# Autodesk Inventor assembly: ExtruderSatoerMirrored
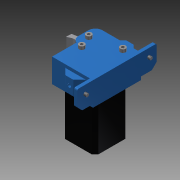
[picture p0: Inventor's stored thumbnail of the model, 180x180]
Saved by Autodesk Inventor 2015 SP1 (Build 190203100, 203)
## iProperties
Created: 2015-05-03
Part Number: ExtruderSatoerMirrored
Document SubType Name: Assembly
Designer: Jack
Author: Jack
## Documents named in this file (13)
- C:\Users\Jack\ownCloud\Projects\CrossBot\InventorModel\Extruder\ExtruderSatoer\ExtruderSatoerLeft\ExtruderSatoerLeft.iam
- C:\Users\Jack\ownCloud\Projects\CrossBot\InventorModel\Extruder\ExtruderSatoer\ExtruderSatoerLeft\ExtruderSatoerBodyLeft.ipt
- C:\Users\Jack\ownCloud\Projects\CrossBot\InventorModel\Extruder\ExtruderSatoer\ExtruderSatoerLeft\ExtruderSatoerMotorMountLeft.ipt
- C:\Users\Jack\ownCloud\Projects\CrossBot\InventorModel\Hardware\Bolts\SHCS\SHCS4\SHCS4x30.ipt
- C:\Users\Jack\ownCloud\Projects\CrossBot\InventorModel\Extruder\ExtruderSatoer\ExtruderSatoerLeft\ExtruderSatoerBearingArmLeft.ipt
- C:\Users\Jack\ownCloud\Projects\CrossBot\InventorModel\Extruder\ExtruderSatoer\ExtruderSatoerLeft\ExtruderSatoerCamLeft.ipt
- C:\Users\Jack\ownCloud\Projects\CrossBot\InventorModel\Extruder\ExtruderSatoer\ExtruderSatoerLeft\ExtruderSatoerCamArmLeft.ipt
- C:\Users\Jack\ownCloud\Projects\CrossBot\InventorModel\Hardware\Bearing\BearingRadialBall\BearingRadialBall624zz.ipt
- C:\Users\Jack\ownCloud\Projects\CrossBot\InventorModel\Hardware\Bolts\SHCS\SHCS4\SHCS4x12.ipt
- C:\Users\Jack\ownCloud\Projects\CrossBot\InventorModel\Hardware\Nuts\Nut4.ipt
- C:\Users\Jack\ownCloud\Projects\CrossBot\InventorModel\Hardware\BoltWashers\BoltWasher4\BoltWasher4x8.iam
- C:\Users\Jack\ownCloud\Projects\CrossBot\InventorModel\Hardware\Bolts\SHCS\SHCS3\SHCS3x12.ipt
- C:\Users\Jack\ownCloud\Projects\CrossBot\InventorModel\Electronics\Motors\StepperMotorNema17x60mm.ipt
## Components (21 placed, 12 different names)
1. ExtruderSatoerBodyLeft:1 — Mate:3, Mate:2, Mate:1, Mate:8, Mate:6, Mate:7, Mate:5, Mate:9, Mate:4, Mate:13, Mate:16, Mate:15, Mate:25, Mate:22, Mate:24, Mate:23
2. ExtruderSatoerMotorMountLeft:1 — Mate:3, Mate:2, Mate:1, Angle:2, Mate:31, Angle:3, Mate:30, Angle:4, Mate:29, Mate:37, Mate:34, Mate:39, Mate:33, Mate:36, Mate:35, Mate:38, Mate:32, Mate:42, Mate:40
3. SHCS4x30:1 — Mate:8, Mate:6, Mate:14, Mate:28
4. SHCS4x30:2 — Mate:7, Mate:5, Mate:12, Mate:26
5. SHCS4x30:3 — Mate:9, Mate:4, Mate:17, Mate:27
6. ExtruderSatoerBearingArmLeft:1 — Mate:13, Mate:12, Mate:11, Mate:10, Mate:19, Mate:18, Mate:21, Angle:1
7. ExtruderSatoerCamLeft:1 — Mate:17, Mate:16
8. ExtruderSatoerCamArmLeft:1 — Mate:15, Mate:14
9. BearingRadialBall624zz:1 — Mate:11, Mate:10
10. SHCS4x12:1 — Mate:19, Mate:18, Mate:20
11. Nut4:1 — Mate:21, Angle:1, Mate:20
12. BoltWasher4x8:1 [sub-assembly] — Mate:25, Mate:22
13. BoltWasher4x8:2 [sub-assembly] — Mate:24, Mate:23
14. Nut4:2 — Angle:2, Mate:31, Mate:26
15. Nut4:3 — Angle:3, Mate:30, Mate:27
16. Nut4:4 — Angle:4, Mate:29, Mate:28
17. SHCS3x12:1 — Mate:37, Mate:34
18. SHCS3x12:2 — Mate:39, Mate:33
19. SHCS3x12:3 — Mate:36, Mate:35
20. SHCS3x12:4 — Mate:38, Mate:32, Mate:41
21. StepperMotorNema17x60mm:1 — Mate:42, Mate:41, Mate:40
## Relationships (46: Mate 42, Angle 4)
- Mate:3: ExtruderSatoerBodyLeft:1 ↔ ExtruderSatoerMotorMountLeft:1
- Mate:2 (0.25 mm): ExtruderSatoerBodyLeft:1 ↔ ExtruderSatoerMotorMountLeft:1
- Mate:1 (0.25 mm): ExtruderSatoerBodyLeft:1 ↔ ExtruderSatoerMotorMountLeft:1
- Mate:8: ExtruderSatoerBodyLeft:1 ↔ SHCS4x30:1
- Mate:6: ExtruderSatoerBodyLeft:1 ↔ SHCS4x30:1
- Mate:7: ExtruderSatoerBodyLeft:1 ↔ SHCS4x30:2
- Mate:5: ExtruderSatoerBodyLeft:1 ↔ SHCS4x30:2
- Mate:9: ExtruderSatoerBodyLeft:1 ↔ SHCS4x30:3
- Mate:4: ExtruderSatoerBodyLeft:1 ↔ SHCS4x30:3
- Mate:13 (0.15 mm): ExtruderSatoerBodyLeft:1 ↔ ExtruderSatoerBearingArmLeft:1
- Mate:12: SHCS4x30:2 ↔ ExtruderSatoerBearingArmLeft:1
- Mate:17: SHCS4x30:3 ↔ ExtruderSatoerCamLeft:1
- Mate:16 (0.15 mm): ExtruderSatoerBodyLeft:1 ↔ ExtruderSatoerCamLeft:1
- Mate:15 (0.15 mm): ExtruderSatoerBodyLeft:1 ↔ ExtruderSatoerCamArmLeft:1
- Mate:14: SHCS4x30:1 ↔ ExtruderSatoerCamArmLeft:1
- Mate:11: ExtruderSatoerBearingArmLeft:1 ↔ BearingRadialBall624zz:1
- Mate:10: ExtruderSatoerBearingArmLeft:1 ↔ BearingRadialBall624zz:1
- Mate:19: ExtruderSatoerBearingArmLeft:1 ↔ SHCS4x12:1
- Mate:18: ExtruderSatoerBearingArmLeft:1 ↔ SHCS4x12:1
- Mate:21: ExtruderSatoerBearingArmLeft:1 ↔ Nut4:1
- Angle:1 (0 deg): ExtruderSatoerBearingArmLeft:1 ↔ Nut4:1
- Mate:20: SHCS4x12:1 ↔ Nut4:1
- Mate:25: ExtruderSatoerBodyLeft:1 ↔ BoltWasher4x8:1
- Mate:22: ExtruderSatoerBodyLeft:1 ↔ BoltWasher4x8:1
- Mate:24: ExtruderSatoerBodyLeft:1 ↔ BoltWasher4x8:2
- Mate:23: ExtruderSatoerBodyLeft:1 ↔ BoltWasher4x8:2
- Angle:2 (0 deg): ExtruderSatoerMotorMountLeft:1 ↔ Nut4:2
- Mate:31: ExtruderSatoerMotorMountLeft:1 ↔ Nut4:2
- Mate:26: SHCS4x30:2 ↔ Nut4:2
- Angle:3 (0 deg): ExtruderSatoerMotorMountLeft:1 ↔ Nut4:3
- Mate:30: ExtruderSatoerMotorMountLeft:1 ↔ Nut4:3
- Mate:27: SHCS4x30:3 ↔ Nut4:3
- Angle:4 (0 deg): ExtruderSatoerMotorMountLeft:1 ↔ Nut4:4
- Mate:29: ExtruderSatoerMotorMountLeft:1 ↔ Nut4:4
- Mate:28: SHCS4x30:1 ↔ Nut4:4
- Mate:37: ExtruderSatoerMotorMountLeft:1 ↔ SHCS3x12:1
- Mate:34: ExtruderSatoerMotorMountLeft:1 ↔ SHCS3x12:1
- Mate:39: ExtruderSatoerMotorMountLeft:1 ↔ SHCS3x12:2
- Mate:33: ExtruderSatoerMotorMountLeft:1 ↔ SHCS3x12:2
- Mate:36: ExtruderSatoerMotorMountLeft:1 ↔ SHCS3x12:3
- Mate:35: ExtruderSatoerMotorMountLeft:1 ↔ SHCS3x12:3
- Mate:38: ExtruderSatoerMotorMountLeft:1 ↔ SHCS3x12:4
- Mate:32: ExtruderSatoerMotorMountLeft:1 ↔ SHCS3x12:4
- Mate:42: ExtruderSatoerMotorMountLeft:1 ↔ StepperMotorNema17x60mm:1
- Mate:41: SHCS3x12:4 ↔ StepperMotorNema17x60mm:1
- Mate:40: ExtruderSatoerMotorMountLeft:1 ↔ StepperMotorNema17x60mm:1
